# Autodesk Inventor assembly: assembled
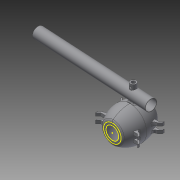
[picture p0: Inventor's stored thumbnail of the model, 180x180]
Saved by Autodesk Inventor 2014 SP2 (Build 180246200, 246)
## iProperties
Created: 2014-11-27
Part Number: assembled
Document SubType Name: Assembly
Designer: No
Author: No
## Documents named in this file (4)
- C:\Users\No\Documents\MAAE3901Design\eggholder\assembled.iam
- C:\Users\No\Documents\MAAE3901Design\eggholder\top-round.ipt
- C:\Users\No\Documents\MAAE3901Design\eggholder\tube.ipt
- C:\Users\No\Documents\MAAE3901Design\eggholder\bottom-round.ipt
## Components (3 placed, 3 different names)
1. top-round:1 — Flush:1, Mate:1, Mate:2, Mate:3, Mate:4, Flush:2, Flush:3
2. tube:1 — Mate:3
3. bottom-round:1 — Mate:4, Flush:2, Flush:3
## Relationships (7: Mate 4, Flush 3)
- Flush:1: top-round:1
- Mate:1: top-round:1
- Mate:2: top-round:1
- Mate:3: top-round:1 ↔ tube:1
- Mate:4: top-round:1 ↔ bottom-round:1
- Flush:2: top-round:1 ↔ bottom-round:1
- Flush:3: top-round:1 ↔ bottom-round:1
